# Autodesk Inventor assembly: Skirt Plug-Panel (Filtered-Mains)
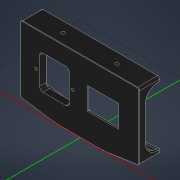
[picture p0: Inventor's stored thumbnail of the model, 180x180]
Saved by Autodesk Inventor 2022 (Build 260153000, 153)
## iProperties
Created: 2022-03-13
Part Number: Skirt Plug-Panel (Filtered-Mains)
Document SubType Name: Assembly
Designer: sleib
Author: sleib
## Documents named in this file (2)
- C:\Users\sleib\Projekte\Voron-2\CAD\Inventor\Skirt Plug-Panel (Filtered-Mains).iam
- C:\Users\sleib\Projekte\Voron-2\CAD\Inventor\Skirt Plug-Panel (Filtered-Mains).ipt
## Components (1 placed, 1 different names)
1. Skirt Plug-Panel (Filtered-Mains):1 — Fluchtend:1, Passend:1, Fluchtend:2
## Relationships (3: Flush 2, Mate 1)
- Fluchtend:1 [Flush]: Skirt Plug-Panel (Filtered-Mains):1
- Passend:1 [Mate]: Skirt Plug-Panel (Filtered-Mains):1
- Fluchtend:2 [Flush] (-58.5 mm): Skirt Plug-Panel (Filtered-Mains):1
